# Autodesk Inventor assembly: Plato Carrete-doble
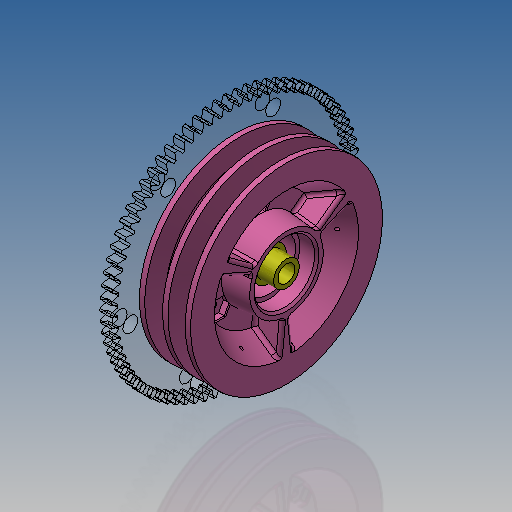
[picture p0: Inventor's stored thumbnail of the model, 512x512]
Saved by Autodesk Inventor 2017 (Build 210142000, 142)
## iProperties
Part Number: Plato Carrete-doble
Material: Genérico
Document SubType Name: Assembly
Designer: Leo
Author: Leo
## Documents named in this file (3)
- C:\Users\Leo\Dropbox\E\Caja Motriz\transmision Engranajes\Plato Carrete-doble.iam
- C:\Users\Leo\Dropbox\E\Caja Motriz\transmision Engranajes\Carrete doble-actuador.ipt
- C:\Users\Leo\Dropbox\E\Caja Motriz\transmision Engranajes\engrane acrílico 2.ipt
## Components (2 placed, 2 different names)
1. Carrete doble-actuador:1 — Nivelación:3
2. engrane acrílico 2:1 — Nivelación:2, Nivelación:1, Nivelación:3
## Relationships (3: Flush 3)
- Nivelación:2 [Flush]: engrane acrílico 2:1
- Nivelación:1 [Flush]: engrane acrílico 2:1
- Nivelación:3 [Flush]: Carrete doble-actuador:1 ↔ engrane acrílico 2:1
